# Autodesk Inventor assembly: ExtendingArm
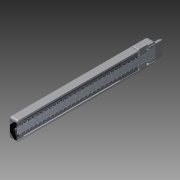
[picture p0: Inventor's stored thumbnail of the model, 180x180]
Saved by Autodesk Inventor 2012 (Build 160160000, 160)
## iProperties
Created: 2011-09-13
Part Number: ExtendingArm
Document SubType Name: Assembly
Designer: KuttaA
Mass: 122.839 g
Surface Area: 790.345 cm^2
Volume: 122.839 cm^3
Density: 1 g/cm^3
Author: KuttaA
## Documents named in this file (7)
- C:\Users\KuttaA\Dropbox\Hexapod Research\Leg Design\ExtendingArm.iam
- C:\Users\KuttaA\Dropbox\Hexapod Research\Leg Design\UpperRobotArm.ipt
- C:\Users\KuttaA\Dropbox\Hexapod Research\Leg Design\UpperArmCap.ipt
- C:\Users\KuttaA\Dropbox\Hexapod Research\Leg Design\LowerArm.ipt
- C:\Users\KuttaA\Dropbox\Hexapod Research\Leg Design\Screw.ipt
- C:\Users\KuttaA\Dropbox\Hexapod Research\Leg Design\InternalKey.ipt
- C:\Users\KuttaA\Dropbox\Hexapod Research\Leg Design\ServoToScrewKey.ipt
## Components (6 placed, 6 different names)
1. UpperRobotArm:1 — Flush:1, Flush:2, Flush:11
2. UpperArmCap:1 — Flush:1
3. LowerArm:1 — Flush:2
4. Screw:1 — Flush:9
5. InternalKey:1 — Flush:11
6. ServoToScrewKey:1 — Flush:9
## Relationships (4: Flush 4)
- Flush:1: UpperRobotArm:1 ↔ UpperArmCap:1
- Flush:2: UpperRobotArm:1 ↔ LowerArm:1
- Flush:9: Screw:1 ↔ ServoToScrewKey:1
- Flush:11: UpperRobotArm:1 ↔ InternalKey:1
## Named parameters: sa_0 = 822.034, sa_1 = 0, sa_2 = 569.438, sa_3 = 757.442, sa_4 = 0, sa_5 = -652.902, sa_6 = 10000
note: some values were not read from the file. Shown as the stored number, unit unknown: "sa_0", "sa_1", "sa_2", "sa_3", "sa_4", "sa_5", "sa_6".
